# Autodesk Inventor assembly: Assembly1
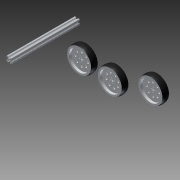
[picture p0: Inventor's stored thumbnail of the model, 180x180]
Saved by Autodesk Inventor 2013 (Build 170138000, 138)
## iProperties
Created: 2013-11-11
Part Number: Assembly1
Document SubType Name: Assembly
Designer: cobrooks
Author: cobrooks
## Documents named in this file (3)
- C:\Users\cobrooks\Documents\GitHub\2013-2014_BlockParty\CAD\Drive\WIMP_mk2\Assembly1.iam
- C:\Users\cobrooks\Documents\GitHub\2013-2014_BlockParty\CAD\COTSParts\Bosch Extrusion\Bosch 20x20.ipt
- C:\Users\cobrooks\Documents\GitHub\2013-2014_BlockParty\CAD\COTSParts\Tetrix\Tetrix wheel 4 in.ipt
## Components (4 placed, 2 different names)
1. Tetrix wheel 4 in:1 — Flush:1, Flush:2, Mate:1, Mate:2, Mate:3
2. Tetrix wheel 4 in:2 — Flush:2
3. Tetrix wheel 4 in:3 — Flush:1
4. Bosch 20x20:1
## Relationships (5: Mate 3, Flush 2)
- Flush:1: Tetrix wheel 4 in:1 ↔ Tetrix wheel 4 in:3
- Flush:2: Tetrix wheel 4 in:1 ↔ Tetrix wheel 4 in:2
- Mate:1: Tetrix wheel 4 in:1
- Mate:2: Tetrix wheel 4 in:1
- Mate:3: Tetrix wheel 4 in:1
